# Autodesk Inventor assembly: konstruktionsprint1
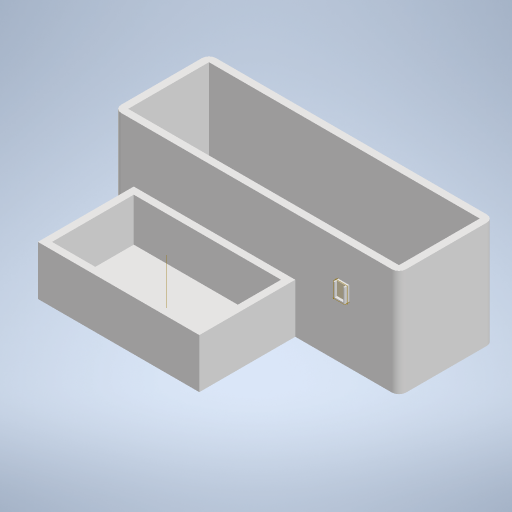
[picture p0: Inventor's stored thumbnail of the model, 512x512]
Saved by Autodesk Inventor 2023 (Build 270158000, 158)
## iProperties
Created: 2025-06-13
Part Number: konstruktionsprint1
Document SubType Name: Assembly
Designer: johan
Author: johan
## Documents named in this file (4)
- C:\Users\johan\OneDrive\Desktop\konstruktionsprint1.iam
- C:\Users\johan\OneDrive\Desktop\beetkasten.ipt
- C:\Users\johan\OneDrive\Desktop\wassertank.ipt
- C:\Users\johan\OneDrive\Desktop\espverkleidung.ipt
## Components (3 placed, 3 different names)
1. beetkasten:1 — Passend:1, Fluchtend:1, Passend:2
2. wassertank:1 — Passend:1, Fluchtend:1
3. espverkleidung:1 — Passend:2
## Relationships (3: Mate 2, Flush 1)
- Passend:1 [Mate]: beetkasten:1 ↔ wassertank:1
- Fluchtend:1 [Flush]: beetkasten:1 ↔ wassertank:1
- Passend:2 [Mate]: beetkasten:1 ↔ espverkleidung:1
